# Autodesk Inventor assembly: Assembly2
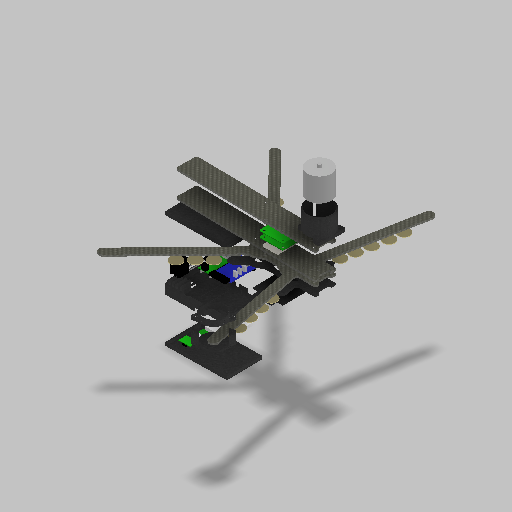
[picture p0: Inventor's stored thumbnail of the model, 512x512]
Saved by Autodesk Inventor 2025.2 (Build 292293000, 293)
## iProperties
Created: 2025-04-10
Part Number: Assembly2
Document SubType Name: Assembly
Designer: joaki
Mass: 215.268 g
Surface Area: 1732.97 cm^2
Volume: 215.268 cm^3
Density: 1 g/cm^3
Author: joaki
## Documents named in this file (13)
- C:\Users\joaki\OneDrive\Dokumenter\Inventor\namo\Full drone.iam
- C:\Users\joaki\OneDrive\Dokumenter\Inventor\namo\Part3.ipt
- C:\Users\joaki\OneDrive\Dokumenter\Inventor\namo\Part4.ipt
- C:\Users\joaki\OneDrive\Dokumenter\Inventor\namo\Part1.ipt
- C:\Users\joaki\OneDrive\Dokumenter\Inventor\namo\CHIP.ipt
- C:\Users\joaki\OneDrive\Dokumenter\Inventor\namo\MOCK DRONE.ipt
- C:\Users\joaki\OneDrive\Dokumenter\Inventor\namo\Part2.ipt
- C:\Users\joaki\OneDrive\Dokumenter\Inventor\namo\top plate.ipt
- C:\Users\joaki\OneDrive\Dokumenter\Inventor\namo\ASSEMBLED SENSOR MODULE.iam
- C:\Users\joaki\OneDrive\Dokumenter\Inventor\namo\pietzo.ipt
- C:\Users\joaki\Downloads\Ringholder.ipt
- C:\Users\joaki\Downloads\NewRing (1).ipt
- C:\Users\joaki\OneDrive\Dokumenter\Inventor\namo\frame top and bottom.ipt
## Components (29 placed, 12 different names)
1. Part3:1 — Rotational:1, Rigid:1, Rotational:2, Rotational:3, Rotational:4
2. Part4:1 — Rotational:1
3. Part1:1 — Rigid:1
4. CHIP:1 — Rotational:2
5. CHIP:2 — Rotational:3
6. MOCK DRONE:1 — Rotational:4, Rigid:2, Mate:1, Mate:2, Mate:3, Mate:4, Mate:5, Mate:6, Mate:7, Mate:8, Mate:9, Mate:10, Mate:11, Mate:12, Mate:13, Mate:14, Mate:15, Mate:16, Mate:17, Rigid:4
7. Part2:1 — Rotational:6
8. top plate:1 — Rotational:6, Rigid:5
9. ASSEMBLED SENSOR MODULE:1 [sub-assembly] — Rigid:2
10. pietzo:1 — Mate:7
11. pietzo:2 — Mate:5
12. pietzo:3 — Mate:16
13. pietzo:4 — Mate:8
14. pietzo:5 — Mate:3
15. pietzo:6 — Mate:4
16. pietzo:7 — Mate:6
17. pietzo:8 — Mate:2
18. pietzo:9 — Mate:1
19. pietzo:10 — Mate:14
20. pietzo:11 — Mate:11
21. pietzo:12 — Mate:15
22. pietzo:13 — Mate:13
23. pietzo:14 — Mate:12
24. pietzo:15 — Mate:10
25. pietzo:16 — Mate:9
26. Ringholder:1 — Mate:17, Rigid:3
27. NewRing (1):1 — Rigid:3
28. frame top and bottom:1 — Rigid:8, Rigid:5
29. frame top and bottom:2 — Rigid:4, Rigid:8
## Relationships (28: Mate 17, WeldJoint 6, RevoluteJoint 5)
- Rotational:1 [RevoluteJoint] (30 mm): Part3:1 ↔ Part4:1
- Rigid:1 [WeldJoint] (30 mm): Part3:1 ↔ Part1:1
- Rotational:2 [RevoluteJoint] (-40 mm): Part3:1 ↔ CHIP:1
- Rotational:3 [RevoluteJoint] (-50 mm): Part3:1 ↔ CHIP:2
- Rotational:4 [RevoluteJoint] (-10 mm): Part3:1 ↔ MOCK DRONE:1
- Rotational:6 [RevoluteJoint] (-20 mm): Part2:1 ↔ top plate:1
- Rigid:2 [WeldJoint] (20 mm): MOCK DRONE:1 ↔ ASSEMBLED SENSOR MODULE:1
- Mate:1 (10 mm): MOCK DRONE:1 ↔ pietzo:9
- Mate:2 (10 mm): MOCK DRONE:1 ↔ pietzo:8
- Mate:3 (10 mm): MOCK DRONE:1 ↔ pietzo:5
- Mate:4 (10 mm): MOCK DRONE:1 ↔ pietzo:6
- Mate:5 (10 mm): MOCK DRONE:1 ↔ pietzo:2
- Mate:6 (10 mm): MOCK DRONE:1 ↔ pietzo:7
- Mate:7 (10 mm): MOCK DRONE:1 ↔ pietzo:1
- Mate:8 (10 mm): MOCK DRONE:1 ↔ pietzo:4
- Mate:9 (10 mm): MOCK DRONE:1 ↔ pietzo:16
- Mate:10 (10 mm): MOCK DRONE:1 ↔ pietzo:15
- Mate:11 (10 mm): MOCK DRONE:1 ↔ pietzo:11
- Mate:12 (10 mm): MOCK DRONE:1 ↔ pietzo:14
- Mate:13 (10 mm): MOCK DRONE:1 ↔ pietzo:13
- Mate:14 (10 mm): MOCK DRONE:1 ↔ pietzo:10
- Mate:15 (10 mm): MOCK DRONE:1 ↔ pietzo:12
- Mate:16 (10 mm): MOCK DRONE:1 ↔ pietzo:3
- Mate:17: MOCK DRONE:1 ↔ Ringholder:1
- Rigid:3 [WeldJoint] (-20 mm): Ringholder:1 ↔ NewRing (1):1
- Rigid:4 [WeldJoint] (-5 mm): MOCK DRONE:1 ↔ frame top and bottom:2
- Rigid:8 [WeldJoint] (-40 mm): frame top and bottom:1 ↔ frame top and bottom:2
- Rigid:5 [WeldJoint] (-20 mm): top plate:1 ↔ frame top and bottom:1
